# Autodesk Inventor assembly: Finished_Basement
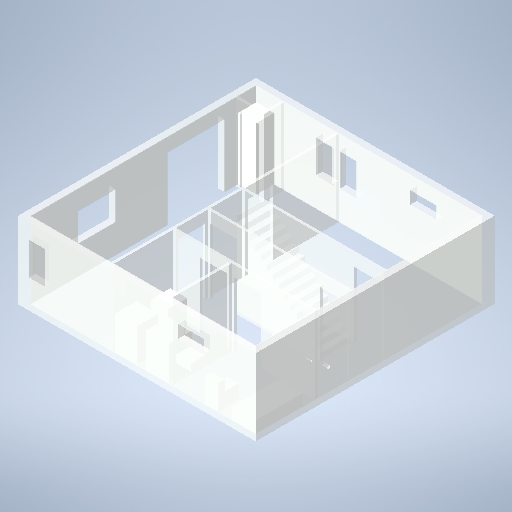
[picture p0: Inventor's stored thumbnail of the model, 512x512]
Saved by Autodesk Inventor 2025.1 (Build 291241020, 241B)
## iProperties
Created: 2023-05-16
Part Number: Finished_Basement
Document SubType Name: Assembly
Designer: Tom
Author: Tom
## Documents named in this file (12)
- C:\Users\Tom\Documents\Inventor\Mobility\Basement\Finished_Basement.iam
- C:\Users\Tom\Documents\Inventor\Mobility\Basement\Exterior_Walls_Of_Finished_Basement.ipt
- C:\Users\Tom\Documents\Inventor\Mobility\Basement\Radon_And_Sump_Systems.ipt
- C:\Users\Tom\Documents\Inventor\Mobility\Basement\Interior_Walls_Of_Finished_Basement.ipt
- C:\Users\Tom\Documents\Inventor\Mobility\Bathtub.ipt
- C:\Users\Tom\Documents\Inventor\Mobility\Bathroom_Sink.ipt
- C:\Users\Tom\Documents\Inventor\Mobility\Toilet.ipt
- C:\Users\Tom\Documents\Inventor\Mobility\Basement\Drier.ipt
- C:\Users\Tom\Documents\Inventor\Mobility\Basement\Washer.ipt
- C:\Users\Tom\Documents\Inventor\Mobility\Basement\Stairs_Between_Finished_Basement_And_First_Floor.ipt
- C:\Users\Tom\Documents\Inventor\Mobility\Basement\Laundry_Room_Sink.ipt
- C:\Users\Tom\Documents\Inventor\Mobility\Basement\Tankless_Water_Heater.ipt
## Components (11 placed, 11 different names)
1. Exterior_Walls_Of_Finished_Basement:1 — Mate:1, Mate:2, Angle:1, Mate:3, Angle:2, Flush:2, Mate:4, Mate:5, Flush:3, Mate:13, Flush:5, Flush:6, Flush:8, Flush:9
2. Radon_And_Sump_Systems:1 — Mate:1, Flush:1, Flush:2
3. Interior_Walls_Of_Finished_Basement:1 — Mate:4, Mate:5, Flush:3, Mate:6, Mate:7, Angle:3, Mate:8, Mate:12, Mate:16, Mate:17, Mate:18, Mate:19, Mate:21, Mate:22, Flush:12, Flush:13, Mate:25, Mate:26, Mate:28, Mate:31
4. Bathtub:1 — Mate:12, Flush:6, Mate:30
5. Bathroom_Sink:1 — Mate:6, Mate:13, Mate:28, Mate:29
6. Toilet:1 — Mate:8, Flush:5, Mate:29
7. Drier:1 — Mate:16, Mate:17, Flush:8
8. Washer:1 — Mate:18, Mate:19, Flush:9
9. Stairs_Between_Finished_Basement_And_First_Floor:1 — Flush:13, Mate:24, Mate:31
10. Laundry_Room_Sink:1 — Mate:21, Mate:22, Flush:12
11. Tankless_Water_Heater:1 — Mate:25, Mate:26
## Relationships (35: Mate 23, Flush 9, Angle 3)
- Mate:1: Exterior_Walls_Of_Finished_Basement:1 ↔ Radon_And_Sump_Systems:1
- Mate:2: Exterior_Walls_Of_Finished_Basement:1
- Angle:1 (90 deg): Exterior_Walls_Of_Finished_Basement:1
- Mate:3: Exterior_Walls_Of_Finished_Basement:1
- Angle:2 (90 deg): Exterior_Walls_Of_Finished_Basement:1
- Flush:1: Radon_And_Sump_Systems:1
- Flush:2: Exterior_Walls_Of_Finished_Basement:1 ↔ Radon_And_Sump_Systems:1
- Mate:4: Exterior_Walls_Of_Finished_Basement:1 ↔ Interior_Walls_Of_Finished_Basement:1
- Mate:5: Exterior_Walls_Of_Finished_Basement:1 ↔ Interior_Walls_Of_Finished_Basement:1
- Flush:3: Exterior_Walls_Of_Finished_Basement:1 ↔ Interior_Walls_Of_Finished_Basement:1
- Mate:6: Interior_Walls_Of_Finished_Basement:1 ↔ Bathroom_Sink:1
- Mate:7: Interior_Walls_Of_Finished_Basement:1
- Angle:3 (90 deg): Interior_Walls_Of_Finished_Basement:1
- Mate:8: Interior_Walls_Of_Finished_Basement:1 ↔ Toilet:1
- Mate:12: Interior_Walls_Of_Finished_Basement:1 ↔ Bathtub:1
- Mate:13 (-914.4 mm): Exterior_Walls_Of_Finished_Basement:1 ↔ Bathroom_Sink:1
- Flush:5: Exterior_Walls_Of_Finished_Basement:1 ↔ Toilet:1
- Flush:6: Exterior_Walls_Of_Finished_Basement:1 ↔ Bathtub:1
- Mate:16: Interior_Walls_Of_Finished_Basement:1 ↔ Drier:1
- Mate:17 (25.4 mm): Interior_Walls_Of_Finished_Basement:1 ↔ Drier:1
- Flush:8: Exterior_Walls_Of_Finished_Basement:1 ↔ Drier:1
- Mate:18: Interior_Walls_Of_Finished_Basement:1 ↔ Washer:1
- Mate:19 (25.4 mm): Interior_Walls_Of_Finished_Basement:1 ↔ Washer:1
- Flush:9: Exterior_Walls_Of_Finished_Basement:1 ↔ Washer:1
- Mate:21: Interior_Walls_Of_Finished_Basement:1 ↔ Laundry_Room_Sink:1
- Mate:22 (101.6 mm): Interior_Walls_Of_Finished_Basement:1 ↔ Laundry_Room_Sink:1
- Flush:12: Interior_Walls_Of_Finished_Basement:1 ↔ Laundry_Room_Sink:1
- Flush:13: Interior_Walls_Of_Finished_Basement:1 ↔ Stairs_Between_Finished_Basement_And_First_Floor:1
- Mate:24 (1028.7 mm): Stairs_Between_Finished_Basement_And_First_Floor:1
- Mate:25: Interior_Walls_Of_Finished_Basement:1 ↔ Tankless_Water_Heater:1
- Mate:26 (25.4 mm): Interior_Walls_Of_Finished_Basement:1 ↔ Tankless_Water_Heater:1
- Mate:28 (114.3 mm): Interior_Walls_Of_Finished_Basement:1 ↔ Bathroom_Sink:1
- Mate:29 (457.2 mm): Bathroom_Sink:1 ↔ Toilet:1
- Mate:30 (19.05 mm): Bathtub:1
- Mate:31: Interior_Walls_Of_Finished_Basement:1 ↔ Stairs_Between_Finished_Basement_And_First_Floor:1
